# Autodesk Inventor assembly: Jetson_Mount
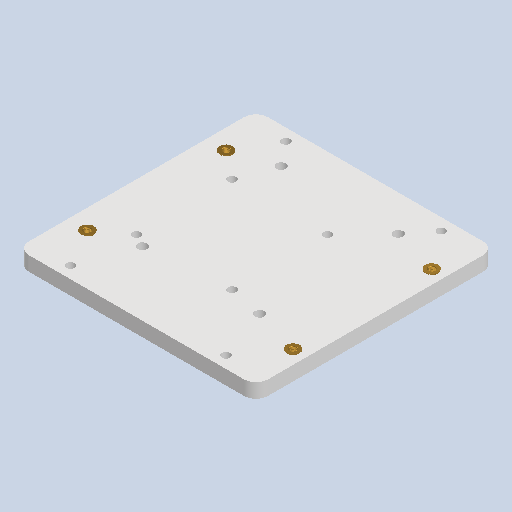
[picture p0: Inventor's stored thumbnail of the model, 512x512]
Saved by Autodesk Inventor 2022 (Build 260153000, 153)
## iProperties
Created: 2022-01-30
Part Number: Jetson_Mount
Document SubType Name: Assembly
Designer: Jorian Brusind
Author: Jorian Brusind
## Documents named in this file (3)
- C:\Users\Jorian Brusind\Documents\GitHub\HyperRail\Inventor Files\Jetson_Mount.iam
- C:\Users\Jorian Brusind\Documents\GitHub\HyperRail\Inventor Files\EboxMounting_Plate.ipt
- C:\Users\Jorian Brusind\Documents\GitHub\HyperRail\Inventor Files\McMaster Files\Heat Inserts\M3-6mm-HeatInsert.ipt
## Components (5 placed, 2 different names)
1. EboxMounting_Plate:1 — Mate:1, Mate:2, Mate:3, Mate:4, Flush:1, Flush:2, Flush:3, Flush:4
2. M3-6mm-HeatInsert:1 — Mate:4, Flush:1
3. M3-6mm-HeatInsert:2 — Mate:2, Flush:2
4. M3-6mm-HeatInsert:3 — Mate:3, Flush:4
5. M3-6mm-HeatInsert:4 — Mate:1, Flush:3
## Relationships (8: Mate 4, Flush 4)
- Mate:1: EboxMounting_Plate:1 ↔ M3-6mm-HeatInsert:4
- Mate:2: EboxMounting_Plate:1 ↔ M3-6mm-HeatInsert:2
- Mate:3: EboxMounting_Plate:1 ↔ M3-6mm-HeatInsert:3
- Mate:4: EboxMounting_Plate:1 ↔ M3-6mm-HeatInsert:1
- Flush:1: EboxMounting_Plate:1 ↔ M3-6mm-HeatInsert:1
- Flush:2: EboxMounting_Plate:1 ↔ M3-6mm-HeatInsert:2
- Flush:3: EboxMounting_Plate:1 ↔ M3-6mm-HeatInsert:4
- Flush:4: EboxMounting_Plate:1 ↔ M3-6mm-HeatInsert:3
